# Autodesk Inventor assembly: XYZ Stage V5
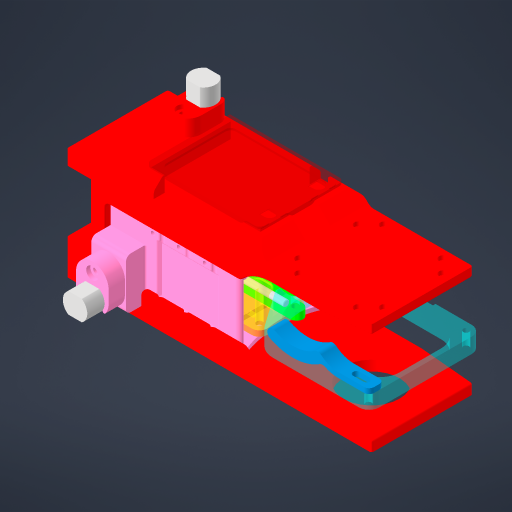
[picture p0: Inventor's stored thumbnail of the model, 512x512]
Saved by Autodesk Inventor 2023.4 (Build 274418000, 418)
## iProperties
Created: 2024-05-20
Part Number: XYZ Stage V5
Document SubType Name: Assembly
Designer: xSibe
Author: xSibe
## Documents named in this file (13)
- C:\.Laptop\.Work\Projects\Project Protocube\1 Autodesk\1 Cubes\XYZ Stage\XYZ Stage V5.iam
- C:\.Laptop\.Work\Projects\Project Protocube\1 Autodesk\1 Cubes\XYZ Stage\Z Stage Body V5.ipt
- C:\.Laptop\.Work\Projects\Project Protocube\1 Autodesk\1 Cubes\XYZ Stage\Z Stage Part V5.ipt
- C:\.Laptop\.Work\Projects\Project Protocube\1 Autodesk\1 Cubes\XYZ Stage\Y Stage Body v5.ipt
- C:\.Laptop\.Work\Projects\Project Protocube\1 Autodesk\1 Cubes\XYZ Stage\Y Stage Part V5.ipt
- C:\.Laptop\.Work\Projects\Project Protocube\1 Autodesk\1 Cubes\XYZ Stage\X Stage Body V5.ipt
- C:\.Laptop\.Work\Projects\Project Protocube\1 Autodesk\1 Cubes\XYZ Stage\X Stage Part V5.ipt
- C:\.Laptop\.Work\Projects\Project Protocube\1 Autodesk\1 Cubes\XYZ Stage\X Stage Clamp V5.ipt
- C:\.Laptop\.Work\Projects\Project Protocube\1 Autodesk\1 Cubes\XYZ Stage\Z Stage Electrical Cover.ipt
- C:\.Laptop\.Work\Projects\Project Protocube\1 Autodesk\1 Cubes\XYZ Stage\Z Stage Motor Clamp V5.ipt
- C:\.Laptop\.Work\Projects\Project Protocube\1 Autodesk\1 Cubes\XYZ Stage\DC Motor.ipt
- C:\.Laptop\.Work\Projects\Project Protocube\1 Autodesk\1 Cubes\XYZ Stage\Y Stage Motor Clamp V5.ipt
- C:\.Laptop\.Work\Projects\Project Protocube\1 Autodesk\1 Cubes\XYZ Stage\X Stage Motor Clamp V5.ipt
## Components (14 placed, 12 different names)
1. DC Motor:1 — Mate:3, Mate:4, Mate:5
2. DC Motor:2 — Mate:6, Mate:7, Mate:8
3. DC Motor:3 — Mate:9, Mate:10, Mate:11
4. Z Stage Body V5:1 — Mate:3, Mate:4, Mate:5, Mate:12
5. Z Stage Part V5:1 — Mate:2, Mate:6, Mate:7, Mate:8, Mate:13
6. Z Stage Electrical Cover:1
7. Z Stage Motor Clamp V5:1 — Mate:12
8. Y Stage Body v5:1 — Mate:2, Mate:9, Mate:10, Mate:11, Mate:14
9. Y Stage Part V5:1
10. Y Stage Motor Clamp V5:1 — Mate:13
11. X Stage Body V5:1
12. X Stage Part V5:1
13. X Stage Clamp V5:1
14. X Stage Motor Clamp V5:1 — Mate:14
## Relationships (13: Mate 13)
- Mate:2 (0.375 mm): Z Stage Part V5:1 ↔ Y Stage Body v5:1
- Mate:3: DC Motor:1 ↔ Z Stage Body V5:1
- Mate:4: DC Motor:1 ↔ Z Stage Body V5:1
- Mate:5: DC Motor:1 ↔ Z Stage Body V5:1
- Mate:6: DC Motor:2 ↔ Z Stage Part V5:1
- Mate:7 (0.075 mm): DC Motor:2 ↔ Z Stage Part V5:1
- Mate:8: DC Motor:2 ↔ Z Stage Part V5:1
- Mate:9: DC Motor:3 ↔ Y Stage Body v5:1
- Mate:10 (0.075 mm): DC Motor:3 ↔ Y Stage Body v5:1
- Mate:11: DC Motor:3 ↔ Y Stage Body v5:1
- Mate:12: Z Stage Body V5:1 ↔ Z Stage Motor Clamp V5:1
- Mate:13: Z Stage Part V5:1 ↔ Y Stage Motor Clamp V5:1
- Mate:14: Y Stage Body v5:1 ↔ X Stage Motor Clamp V5:1
